# Autodesk Inventor assembly: MG-Grundplatte
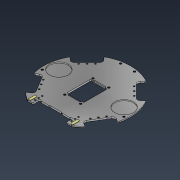
[picture p0: Inventor's stored thumbnail of the model, 180x180]
Saved by Autodesk Inventor 2022.1 (Build 261234020, 234B)
## iProperties
Part Number: MG-Grundplatte
Material: Generisch
Document SubType Name: Assembly
Designer: rYan
Mass: 128.652 g
Surface Area: 395.086 cm^2
Volume: 47.6131 cm^3
Density: 2.70203 g/cm^3
Author: rYan
## Documents named in this file (4)
- D:\TIGERsGIT\Hardware\mechanik\2020\Inventor\Robot\MG-Grundplatte.iam
- D:\TIGERsGIT\Hardware\mechanik\2020\Inventor\Robot\Grundplatte.ipt
- D:\TIGERsGIT\Hardware\mechanik\2020\Inventor\Robot\Dribbler\Dribblerdaempfer Unten.ipt
- D:\TIGERsGIT\Hardware\mechanik\2020\Inventor\Robot\Dribbler\Dribblerdaempfer Unten V2.ipt
## Components (5 placed, 3 different names)
1. Grundplatte:1 — Fluchtend:1, Passend:1, Passend:2, Passend:3, Passend:4, Tangential:1, Tangential:2, Passend:5, Passend:6, Passend:7, Passend:8, Passend:9, Passend:10, Tangential:3, Tangential:4
2. Dribblerdaempfer Unten:1 — Passend:3, Tangential:2, Passend:6
3. Dribblerdaempfer Unten:2 — Passend:4, Tangential:1, Passend:5
4. Dribblerdaempfer Unten V2:1 — Passend:7, Passend:10, Tangential:3
5. Dribblerdaempfer Unten V2:2 — Passend:8, Passend:9, Tangential:4
## Relationships (15: Mate 10, Tangent 4, Flush 1)
- Fluchtend:1 [Flush]: Grundplatte:1
- Passend:1 [Mate]: Grundplatte:1
- Passend:2 [Mate]: Grundplatte:1
- Passend:3 [Mate]: Grundplatte:1 ↔ Dribblerdaempfer Unten:1
- Passend:4 [Mate]: Grundplatte:1 ↔ Dribblerdaempfer Unten:2
- Tangential:1: Grundplatte:1 ↔ Dribblerdaempfer Unten:2
- Tangential:2: Grundplatte:1 ↔ Dribblerdaempfer Unten:1
- Passend:5 [Mate]: Grundplatte:1 ↔ Dribblerdaempfer Unten:2
- Passend:6 [Mate]: Grundplatte:1 ↔ Dribblerdaempfer Unten:1
- Passend:7 [Mate]: Grundplatte:1 ↔ Dribblerdaempfer Unten V2:1
- Passend:8 [Mate]: Grundplatte:1 ↔ Dribblerdaempfer Unten V2:2
- Passend:9 [Mate]: Grundplatte:1 ↔ Dribblerdaempfer Unten V2:2
- Passend:10 [Mate]: Grundplatte:1 ↔ Dribblerdaempfer Unten V2:1
- Tangential:3: Grundplatte:1 ↔ Dribblerdaempfer Unten V2:1
- Tangential:4: Grundplatte:1 ↔ Dribblerdaempfer Unten V2:2
